# Autodesk Inventor assembly: chassisstructure
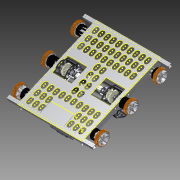
[picture p0: Inventor's stored thumbnail of the model, 180x180]
Saved by Autodesk Inventor 2014 SP1 (Build 180222100, 222)
## iProperties
Created: 2014-01-04
Part Number: chassisstructure
Document SubType Name: Assembly
Designer: Arpan
Mass: 5943.64 g
Surface Area: 26488.1 cm^2
Volume: 5337.4 cm^3
Density: 1.11358 g/cm^3
Author: Arpan
## Documents named in this file (16)
- C:\Users\Arpan\Documents\GitHub\2014buildCAD\chassisdrivetrain\chassis light\chassisstructure.iam
- C:\Users\Arpan\Documents\GitHub\2014buildCAD\chassisdrivetrain\chassis light\chassis front back rail.ipt
- C:\Users\Arpan\Documents\GitHub\2014buildCAD\chassisdrivetrain\chassis light\chassis side rail.ipt
- C:\Users\Arpan\Documents\GitHub\2014buildCAD\chassisdrivetrain\gearbot\3cimgearbox.iam
- C:\Users\Arpan\Documents\GitHub\2014buildCAD\chassisdrivetrain\chassis light\COTS items\center wheel assembly.iam
- C:\Users\Arpan\Documents\GitHub\2014buildCAD\chassisdrivetrain\chassis light\COTS items\.5 inch bearing pretend its hex.ipt
- C:\Users\Arpan\Documents\GitHub\2014buildCAD\chassisdrivetrain\chassis light\4.5 hex shaft.ipt
- C:\Users\Arpan\Documents\GitHub\2014buildCAD\chassisdrivetrain\chassis light\COTS items\front wheels.iam
- C:\Users\Arpan\Documents\GitHub\2014buildCAD\chassisdrivetrain\chassis light\COTS items\back wheels.iam
- C:\Users\Arpan\Documents\GitHub\2014buildCAD\chassisdrivetrain\chassis light\COTS items\DBK_42ToothPulley V2.iam
- C:\Users\Arpan\Documents\GitHub\2014buildCAD\chassisdrivetrain\chassis light\3d printed items\back wheel spacer.ipt
- C:\Users\Arpan\Documents\GitHub\2014buildCAD\chassisdrivetrain\chassis light\PVC pipe spacer.ipt
- C:\Users\Arpan\Documents\GitHub\2014buildCAD\chassisdrivetrain\chassis light\PVC pipe spacer center wheels.ipt
- C:\Users\Arpan\Documents\GitHub\2014buildCAD\chassisdrivetrain\chassis light\baseplate.ipt
- C:\Users\Arpan\Documents\GitHub\2014buildCAD\chassisdrivetrain\chassis light\battery mount.ipt
- C:\Users\Arpan\Documents\GitHub\2014buildCAD\electrical\ELEC_Battery_NP18-12B.iam
## Components (37 placed, 15 different names)
1. chassis front back rail:1 — Mate:5, Flush:4, Angle:1, Flush:5, Mate:65, Mate:66
2. chassis side rail:1 — Mate:3, Mate:4, Flush:2, Mate:5, Flush:4, Mate:6, Mate:7, Mate:14, Mate:15, Mate:16, Mate:17, Mate:18, Mate:19, Mate:20, Mate:29, Mate:56, Mate:58, Mate:62, Mate:67
3. chassis front back rail:2 — Flush:1, Mate:1, Mate:2, Mate:3, Mate:4, Flush:2, Flush:5, Flush:24
4. chassis side rail:2 — Flush:1, Mate:1, Mate:2, Mate:8, Mate:9, Mate:21, Mate:22, Mate:23, Mate:24, Mate:25, Mate:26, Mate:27, Mate:28, Angle:3, Mate:54, Mate:60, Mate:64, Flush:25
5. 3cimgearbox:1 [sub-assembly] — Mate:6, Mate:7, Angle:1, Angle:2, Flush:7, Mate:12, Mate:13, Mate:61
6. 3cimgearbox:2 [sub-assembly] — Mate:8, Mate:9, Angle:2, Flush:6, Mate:10, Mate:11, Mate:63
7. center wheel assembly:1 [sub-assembly] — Flush:6, Mate:10, Mate:11, Flush:17, Flush:18, Flush:22
8. center wheel assembly:2 [sub-assembly] — Flush:7, Mate:12, Mate:13, Flush:21, Flush:23
9. .5 inch bearing pretend its hex:1 — Mate:16, Mate:17
10. .5 inch bearing pretend its hex:2 — Mate:14, Mate:15, Mate:30
11. .5 inch bearing pretend its hex:3 — Mate:19, Mate:29
12. .5 inch bearing pretend its hex:4 — Mate:18, Mate:20, Mate:31
13. .5 inch bearing pretend its hex:5 — Mate:21, Mate:24, Mate:33
14. .5 inch bearing pretend its hex:6 — Mate:22, Mate:23
15. .5 inch bearing pretend its hex:7 — Mate:25, Mate:26, Mate:32
16. .5 inch bearing pretend its hex:8 — Mate:27, Mate:28
17. 4.5 hex shaft:1 — Mate:30, Flush:9, Flush:13, Mate:36, Mate:37, Mate:55
18. 4.5 hex shaft:2 — Mate:31, Flush:9, Flush:15, Mate:40, Mate:41, Mate:57
19. 4.5 hex shaft:3 — Mate:32, Flush:11, Mate:34, Mate:35, Angle:3, Flush:19, Mate:59
20. 4.5 hex shaft:4 — Flush:11, Mate:33, Mate:38, Mate:39, Flush:20, Mate:53
21. front wheels:1 [sub-assembly] — Mate:34, Mate:35, Flush:17, Flush:19
22. front wheels:2 [sub-assembly] — Flush:13, Mate:36, Mate:37, Flush:21
23. back wheels:1 [sub-assembly] — Flush:15, Mate:40, Mate:41, Mate:42, Mate:43, Mate:44, Mate:48, Mate:49
24. back wheels:2 [sub-assembly] — Mate:38, Mate:39, Mate:45, Mate:46, Flush:18, Flush:20, Mate:51, Mate:52
25. DBK_42ToothPulley V2:1 [sub-assembly] — Mate:42, Mate:43, Mate:44, Flush:23, Mate:47
26. DBK_42ToothPulley V2:2 [sub-assembly] — Mate:45, Mate:46, Flush:22, Mate:50
27. back wheel spacer:1 — Mate:47, Mate:48, Mate:49
28. back wheel spacer:2 — Mate:50, Mate:51, Mate:52
29. PVC pipe spacer:1 — Mate:55, Mate:56
30. PVC pipe spacer:2 — Mate:57, Mate:58
31. PVC pipe spacer:3 — Mate:53, Mate:54
32. PVC pipe spacer:4 — Mate:59, Mate:60
33. PVC pipe spacer center wheels:1 — Mate:61, Mate:62
34. PVC pipe spacer center wheels:2 — Mate:63, Mate:64
35. baseplate:1 — Mate:65, Flush:24, Flush:25, Mate:69
36. battery mount:1 — Mate:66, Mate:67, Mate:68
37. ELEC_Battery_NP18-12B:1 [sub-assembly] — Mate:68, Mate:69
## Relationships (91: Mate 69, Flush 19, Angle 3)
- Flush:1 (-86.36 mm): chassis front back rail:2 ↔ chassis side rail:2
- Mate:1: chassis front back rail:2 ↔ chassis side rail:2
- Mate:2: chassis front back rail:2 ↔ chassis side rail:2
- Mate:3: chassis side rail:1 ↔ chassis front back rail:2
- Mate:4: chassis side rail:1 ↔ chassis front back rail:2
- Flush:2 (-86.36 mm): chassis side rail:1 ↔ chassis front back rail:2
- Mate:5: chassis front back rail:1 ↔ chassis side rail:1
- Flush:4: chassis front back rail:1 ↔ chassis side rail:1
- Mate:6: chassis side rail:1 ↔ 3cimgearbox:1
- Mate:7: chassis side rail:1 ↔ 3cimgearbox:1
- Angle:1 (0 deg): chassis front back rail:1 ↔ 3cimgearbox:1
- Mate:8: chassis side rail:2 ↔ 3cimgearbox:2
- Mate:9: chassis side rail:2 ↔ 3cimgearbox:2
- Angle:2 (0 deg): 3cimgearbox:1 ↔ 3cimgearbox:2
- Flush:5: chassis front back rail:1 ↔ chassis front back rail:2
- Flush:6: 3cimgearbox:2 ↔ center wheel assembly:1
- Mate:10: 3cimgearbox:2 ↔ center wheel assembly:1
- Mate:11: 3cimgearbox:2 ↔ center wheel assembly:1
- Flush:7: 3cimgearbox:1 ↔ center wheel assembly:2
- Mate:12: 3cimgearbox:1 ↔ center wheel assembly:2
- Mate:13: 3cimgearbox:1 ↔ center wheel assembly:2
- Mate:14: chassis side rail:1 ↔ .5 inch bearing pretend its hex:2
- Mate:15: chassis side rail:1 ↔ .5 inch bearing pretend its hex:2
- Mate:16: chassis side rail:1 ↔ .5 inch bearing pretend its hex:1
- Mate:17: chassis side rail:1 ↔ .5 inch bearing pretend its hex:1
- Mate:18: chassis side rail:1 ↔ .5 inch bearing pretend its hex:4
- Mate:19: chassis side rail:1 ↔ .5 inch bearing pretend its hex:3
- Mate:20: chassis side rail:1 ↔ .5 inch bearing pretend its hex:4
- Mate:21: chassis side rail:2 ↔ .5 inch bearing pretend its hex:5
- Mate:22: chassis side rail:2 ↔ .5 inch bearing pretend its hex:6
- Mate:23: chassis side rail:2 ↔ .5 inch bearing pretend its hex:6
- Mate:24: chassis side rail:2 ↔ .5 inch bearing pretend its hex:5
- Mate:25: chassis side rail:2 ↔ .5 inch bearing pretend its hex:7
- Mate:26: chassis side rail:2 ↔ .5 inch bearing pretend its hex:7
- Mate:27: chassis side rail:2 ↔ .5 inch bearing pretend its hex:8
- Mate:28: chassis side rail:2 ↔ .5 inch bearing pretend its hex:8
- Mate:29: chassis side rail:1 ↔ .5 inch bearing pretend its hex:3
- Mate:30: .5 inch bearing pretend its hex:2 ↔ 4.5 hex shaft:1
- Mate:31: .5 inch bearing pretend its hex:4 ↔ 4.5 hex shaft:2
- Flush:9: 4.5 hex shaft:1 ↔ 4.5 hex shaft:2
- Mate:32: .5 inch bearing pretend its hex:7 ↔ 4.5 hex shaft:3
- Flush:11: 4.5 hex shaft:3 ↔ 4.5 hex shaft:4
- Mate:33: .5 inch bearing pretend its hex:5 ↔ 4.5 hex shaft:4
- Mate:34: 4.5 hex shaft:3 ↔ front wheels:1
- Mate:35: 4.5 hex shaft:3 ↔ front wheels:1
- Flush:13: 4.5 hex shaft:1 ↔ front wheels:2
- Mate:36: 4.5 hex shaft:1 ↔ front wheels:2
- Mate:37: 4.5 hex shaft:1 ↔ front wheels:2
- Mate:38: 4.5 hex shaft:4 ↔ back wheels:2
- Mate:39: 4.5 hex shaft:4 ↔ back wheels:2
- Flush:15: 4.5 hex shaft:2 ↔ back wheels:1
- Mate:40: 4.5 hex shaft:2 ↔ back wheels:1
- Mate:41: 4.5 hex shaft:2 ↔ back wheels:1
- Mate:42: back wheels:1 ↔ DBK_42ToothPulley V2:1
- Mate:43: back wheels:1 ↔ DBK_42ToothPulley V2:1
- Mate:44: back wheels:1 ↔ DBK_42ToothPulley V2:1
- Mate:45: back wheels:2 ↔ DBK_42ToothPulley V2:2
- Mate:46: back wheels:2 ↔ DBK_42ToothPulley V2:2
- Flush:17: center wheel assembly:1 ↔ front wheels:1
- Flush:18: center wheel assembly:1 ↔ back wheels:2
- Angle:3 (0 deg): chassis side rail:2 ↔ 4.5 hex shaft:3
- Flush:19: 4.5 hex shaft:3 ↔ front wheels:1
- Flush:20: 4.5 hex shaft:4 ↔ back wheels:2
- Flush:21: center wheel assembly:2 ↔ front wheels:2
- Flush:22: center wheel assembly:1 ↔ DBK_42ToothPulley V2:2
- Flush:23: center wheel assembly:2 ↔ DBK_42ToothPulley V2:1
- Mate:47: DBK_42ToothPulley V2:1 ↔ back wheel spacer:1
- Mate:48: back wheels:1 ↔ back wheel spacer:1
- Mate:49: back wheels:1 ↔ back wheel spacer:1
- Mate:50: DBK_42ToothPulley V2:2 ↔ back wheel spacer:2
- Mate:51: back wheels:2 ↔ back wheel spacer:2
- Mate:52: back wheels:2 ↔ back wheel spacer:2
- Mate:53: 4.5 hex shaft:4 ↔ PVC pipe spacer:3
- Mate:54: chassis side rail:2 ↔ PVC pipe spacer:3
- Mate:55: 4.5 hex shaft:1 ↔ PVC pipe spacer:1
- Mate:56: chassis side rail:1 ↔ PVC pipe spacer:1
- Mate:57: 4.5 hex shaft:2 ↔ PVC pipe spacer:2
- Mate:58: chassis side rail:1 ↔ PVC pipe spacer:2
- Mate:59: 4.5 hex shaft:3 ↔ PVC pipe spacer:4
- Mate:60: chassis side rail:2 ↔ PVC pipe spacer:4
- Mate:61: 3cimgearbox:1 ↔ PVC pipe spacer center wheels:1
- Mate:62: chassis side rail:1 ↔ PVC pipe spacer center wheels:1
- Mate:63: 3cimgearbox:2 ↔ PVC pipe spacer center wheels:2
- Mate:64: chassis side rail:2 ↔ PVC pipe spacer center wheels:2
- Mate:65: chassis front back rail:1 ↔ baseplate:1
- Flush:24: chassis front back rail:2 ↔ baseplate:1
- Flush:25: chassis side rail:2 ↔ baseplate:1
- Mate:66: chassis front back rail:1 ↔ battery mount:1
- Mate:67 (49.53 mm): chassis side rail:1 ↔ battery mount:1
- Mate:68: battery mount:1 ↔ ELEC_Battery_NP18-12B:1
- Mate:69: baseplate:1 ↔ ELEC_Battery_NP18-12B:1
